# Autodesk Inventor assembly: Carriage_Link_COG
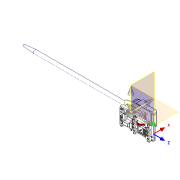
[picture p0: Inventor's stored thumbnail of the model, 180x180]
Saved by Autodesk Inventor 2022 (Build 260153000, 153)
## iProperties
Created: 2022-10-18
Part Number: Carriage_Link_COG
Document SubType Name: Assembly
Designer: alexw
Mass: 599.264 g
Surface Area: 1993.78 cm^2
Volume: 535.454 cm^3
Density: 1.11917 g/cm^3
Author: alexw
## Documents named in this file (22)
- C:\Users\alexw\Documents\Inventor\Projects\03_CurrentProjects\MasterThesis\PSM_V1_Rillenkugellager\COG\Carriage_Link_COG.iam
- C:\Users\alexw\Documents\Inventor\Projects\03_CurrentProjects\MasterThesis\PSM_V1_Rillenkugellager\Ueberarbeiteter DaVincikopf\Fuehrungsgrundplatte_V3.ipt
- C:\Users\alexw\Documents\Inventor\Projects\03_CurrentProjects\MasterThesis\PSM_V1_Rillenkugellager\Ueberarbeiteter DaVincikopf\JX BLS-HV7146MG.iam
- C:\Users\alexw\Documents\Inventor\Projects\03_CurrentProjects\MasterThesis\PSM_V1_Rillenkugellager\Ueberarbeiteter DaVincikopf\Op_dev_gehäuse.ipt
- C:\Users\alexw\Documents\Inventor\Projects\03_CurrentProjects\MasterThesis\PSM_V1_Rillenkugellager\Ueberarbeiteter DaVincikopf\Op_dev_stange.ipt
- C:\Users\alexw\Documents\Inventor\Projects\03_CurrentProjects\MasterThesis\PSM_V1_Rillenkugellager\Ueberarbeiteter DaVincikopf\Oberteil_servoplatte.ipt
- C:\Users\alexw\Documents\Inventor\Projects\03_CurrentProjects\MasterThesis\PSM_V1_Rillenkugellager\ContentCenter\de-DE\ISO 4762(2)\ISO 4762 - M4 x 30ISO.ipt
- C:\Users\alexw\Documents\Inventor\Projects\03_CurrentProjects\MasterThesis\PSM_V1_Rillenkugellager\ContentCenter\de-DE\ISO 4762(2)\ISO 4762 - M3 x 12ISO.ipt
- C:\Users\alexw\Documents\Inventor\Projects\03_CurrentProjects\MasterThesis\PSM_V1_Rillenkugellager\Ueberarbeiteter DaVincikopf\daVinciTool_Aufnahme.ipt
- C:\Users\alexw\Documents\Inventor\Projects\03_CurrentProjects\MasterThesis\PSM_V1_Rillenkugellager\Ueberarbeiteter DaVincikopf\daVinciTool_Aufnahme_ClutchPart.ipt
- C:\Users\alexw\Documents\Inventor\Projects\03_CurrentProjects\MasterThesis\PSM_V1_Rillenkugellager\Ueberarbeiteter DaVincikopf\daVincihead_Sled_ToolAufnahmeBuegel.ipt
- C:\Users\alexw\Documents\Inventor\Projects\03_CurrentProjects\MasterThesis\PSM_V1_Rillenkugellager\Ueberarbeiteter DaVincikopf\daVincihead_Sled_ToolAufnahmeBuegel_38mm.ipt
- C:\Users\alexw\Documents\Inventor\Projects\03_CurrentProjects\MasterThesis\PSM_V1_Rillenkugellager\Ueberarbeiteter DaVincikopf\3mmSchaft_50m.ipt
- C:\Users\alexw\Documents\Inventor\Projects\03_CurrentProjects\MasterThesis\PSM_V1_Rillenkugellager\Ueberarbeiteter DaVincikopf\3mmSchaft_63mm.ipt
- C:\Users\alexw\Documents\Inventor\Projects\03_CurrentProjects\MasterThesis\PSM_V1_Rillenkugellager\Ueberarbeiteter DaVincikopf\Fuehrungsrollen_Assembly.iam
- C:\Users\alexw\Documents\Inventor\Projects\03_CurrentProjects\MasterThesis\PSM_V1_Rillenkugellager\ContentCenter\de-DE\ISO 4762(2)\ISO 4762 - M3 x 10ISO.ipt
- C:\Users\alexw\Documents\Inventor\Projects\03_CurrentProjects\MasterThesis\PSM_V1_Rillenkugellager\Maschinenbauteil\spur_gear_1_30_6_6.ipt
- C:\Users\alexw\Documents\Inventor\Projects\03_CurrentProjects\MasterThesis\PSM_V1_Rillenkugellager\Ueberarbeiteter DaVincikopf\daVinciHead_HITEC_Assembly.iam
- C:\Users\alexw\Documents\Inventor\Projects\03_CurrentProjects\MasterThesis\PSM_V1_Rillenkugellager\Ueberarbeiteter DaVincikopf\Anpresspinns_Assembly.iam
- C:\Users\alexw\Documents\Inventor\Projects\03_CurrentProjects\MasterThesis\PSM_V1_Rillenkugellager\ContentCenter\de-DE\ISO 4762(2)\ISO 4762 - M4 x 12ISO.ipt
- C:\Users\alexw\Documents\Inventor\Projects\03_CurrentProjects\MasterThesis\PSM_V1_Rillenkugellager\ContentCenter\de-DE\ISO 10642(1)\ISO 10642 - M3 x  8.ipt
- C:\Users\alexw\Documents\Inventor\Projects\03_CurrentProjects\MasterThesis\PSM_V1_Rillenkugellager\ContentCenter\de-DE\ISO 4762(2)\ISO 4762 - M3 x 8ISO.ipt
## Components (46 placed, 21 different names)
1. Fuehrungsgrundplatte_V3:1 — Passend:95, Winkel:1, Passend:97
2. JX BLS-HV7146MG:1 [sub-assembly]
3. Op_dev_gehäuse:1
4. Op_dev_stange:1
5. Oberteil_servoplatte:1
6. ISO 4762 M4 x 30:1
7. ISO 4762 M4 x 30:2
8. ISO 4762 M3 x 12:1
9. ISO 4762 M3 x 12:2
10. ISO 4762 M3 x 12:3
11. ISO 4762 M3 x 12:4
12. daVinciTool_Aufnahme:1
13. daVinciTool_Aufnahme_ClutchPart:1
14. daVincihead_Sled_ToolAufnahmeBuegel:1 — Passend:96
15. daVincihead_Sled_ToolAufnahmeBuegel_38mm:1
16. 3mmSchaft_50m:1
17. 3mmSchaft_63mm:1
18. ISO 4762 M3 x 12:5
19. ISO 4762 M3 x 12:6
20. ISO 4762 M3 x 12:7
21. ISO 4762 M3 x 12:8
22. Fuehrungsrollen_Assembly:1 [sub-assembly]
23. Fuehrungsrollen_Assembly:2 [sub-assembly]
24. Fuehrungsrollen_Assembly:3 [sub-assembly]
25. ISO 4762 M3 x 10:1
26. ISO 4762 M3 x 10:2
27. ISO 4762 M3 x 10:3
28. ISO 4762 M3 x 10:4
29. ISO 4762 M3 x 10:5
30. ISO 4762 M3 x 10:6
31. spur_gear_1_30_6_6:1
32. daVinciHead_HITEC_Assembly:1 [sub-assembly]
33. daVinciHead_HITEC_Assembly:2 [sub-assembly]
34. daVinciHead_HITEC_Assembly:3 [sub-assembly]
35. daVinciHead_HITEC_Assembly:4 [sub-assembly]
36. Anpresspinns_Assembly:1 [sub-assembly]
37. Anpresspinns_Assembly:2 [sub-assembly]
38. Anpresspinns_Assembly:3 [sub-assembly]
39. Anpresspinns_Assembly:4 [sub-assembly]
40. ISO 4762 M4 x 12:1
41. 3mmSchaft_63mm:2
42. ISO 10642 M3x8:1
43. ISO 4762 M3 x 8:1
44. ISO 4762 M3 x 8:2
45. ISO 4762 M3 x 8:3
46. ISO 4762 M3 x 8:4
## Relationships (104: Mate 97, Flush 5, RevoluteJoint 1, Angle 1)
- [Flush] (-5 mm): Fuehrungsgrundplatte_V3:1 ↔ JX BLS-HV7146MG:1
- [Mate]: Fuehrungsgrundplatte_V3:1 ↔ JX BLS-HV7146MG:1
- [Mate]: Fuehrungsgrundplatte_V3:1 ↔ JX BLS-HV7146MG:1
- [RevoluteJoint]: Op_dev_gehäuse:1 ↔ Op_dev_stange:1
- [Mate]: Fuehrungsgrundplatte_V3:1 ↔ Oberteil_servoplatte:1
- [Flush]: Fuehrungsgrundplatte_V3:1 ↔ Oberteil_servoplatte:1
- [Mate]: Fuehrungsgrundplatte_V3:1 ↔ ISO 4762 M4 x 30:1
- [Mate]: Fuehrungsgrundplatte_V3:1 ↔ ISO 4762 M4 x 30:2
- [Mate]: Oberteil_servoplatte:1 ↔ ISO 4762 M3 x 12:1
- [Mate]: Oberteil_servoplatte:1 ↔ ISO 4762 M3 x 12:1
- [Mate]: Oberteil_servoplatte:1 ↔ ISO 4762 M3 x 12:2
- [Mate]: Oberteil_servoplatte:1 ↔ ISO 4762 M3 x 12:2
- [Mate]: Oberteil_servoplatte:1 ↔ ISO 4762 M3 x 12:3
- [Mate]: Oberteil_servoplatte:1 ↔ ISO 4762 M3 x 12:3
- [Mate]: Oberteil_servoplatte:1 ↔ ISO 4762 M3 x 12:4
- [Mate]: Oberteil_servoplatte:1 ↔ ISO 4762 M3 x 12:4
- [Mate] (-6.043 mm): Op_dev_gehäuse:1 ↔ daVinciTool_Aufnahme:1
- [Mate]: Op_dev_gehäuse:1 ↔ daVinciTool_Aufnahme:1
- [Flush]: daVinciTool_Aufnahme:1 ↔ daVinciTool_Aufnahme_ClutchPart:1
- [Mate]: Oberteil_servoplatte:1 ↔ daVincihead_Sled_ToolAufnahmeBuegel:1
- [Mate]: Oberteil_servoplatte:1 ↔ daVincihead_Sled_ToolAufnahmeBuegel_38mm:1
- [Mate]: daVincihead_Sled_ToolAufnahmeBuegel:1 ↔ 3mmSchaft_63mm:1
- [Mate]: daVincihead_Sled_ToolAufnahmeBuegel_38mm:1 ↔ 3mmSchaft_50m:1
- [Mate]: daVincihead_Sled_ToolAufnahmeBuegel_38mm:1 ↔ 3mmSchaft_50m:1
- [Mate]: daVinciTool_Aufnahme:1 ↔ 3mmSchaft_63mm:1
- [Mate]: Oberteil_servoplatte:1 ↔ daVinciTool_Aufnahme:1
- [Mate]: daVincihead_Sled_ToolAufnahmeBuegel_38mm:1 ↔ ISO 4762 M3 x 12:5
- [Mate]: Oberteil_servoplatte:1 ↔ ISO 4762 M3 x 12:5
- [Mate]: daVincihead_Sled_ToolAufnahmeBuegel_38mm:1 ↔ ISO 4762 M3 x 12:6
- [Mate]: Oberteil_servoplatte:1 ↔ ISO 4762 M3 x 12:6
- [Mate]: daVincihead_Sled_ToolAufnahmeBuegel:1 ↔ ISO 4762 M3 x 12:7
- [Mate]: Oberteil_servoplatte:1 ↔ ISO 4762 M3 x 12:7
- [Mate]: daVincihead_Sled_ToolAufnahmeBuegel:1 ↔ ISO 4762 M3 x 12:8
- [Mate]: Oberteil_servoplatte:1 ↔ ISO 4762 M3 x 12:8
- [Mate]: Oberteil_servoplatte:1 ↔ daVincihead_Sled_ToolAufnahmeBuegel_38mm:1
- [Mate]: Oberteil_servoplatte:1 ↔ daVincihead_Sled_ToolAufnahmeBuegel_38mm:1
- [Mate]: Oberteil_servoplatte:1 ↔ daVincihead_Sled_ToolAufnahmeBuegel:1
- [Mate]: Fuehrungsgrundplatte_V3:1 ↔ Fuehrungsrollen_Assembly:1
- [Mate]: Fuehrungsgrundplatte_V3:1 ↔ Fuehrungsrollen_Assembly:1
- [Mate]: Fuehrungsgrundplatte_V3:1 ↔ Fuehrungsrollen_Assembly:1
- [Mate]: Fuehrungsgrundplatte_V3:1 ↔ Fuehrungsrollen_Assembly:2
- [Mate]: Fuehrungsgrundplatte_V3:1 ↔ Fuehrungsrollen_Assembly:2
- [Mate]: Fuehrungsgrundplatte_V3:1 ↔ Fuehrungsrollen_Assembly:2
- [Mate]: Fuehrungsgrundplatte_V3:1 ↔ Fuehrungsrollen_Assembly:3
- [Mate]: Fuehrungsgrundplatte_V3:1 ↔ Fuehrungsrollen_Assembly:3
- [Mate]: Fuehrungsgrundplatte_V3:1 ↔ Fuehrungsrollen_Assembly:3
- [Mate]: Fuehrungsrollen_Assembly:1 ↔ ISO 4762 M3 x 10:1
- [Mate]: Fuehrungsrollen_Assembly:1 ↔ ISO 4762 M3 x 10:1
- [Mate]: Fuehrungsrollen_Assembly:1 ↔ ISO 4762 M3 x 10:2
- [Mate]: Fuehrungsrollen_Assembly:1 ↔ ISO 4762 M3 x 10:2
- [Mate]: Fuehrungsrollen_Assembly:2 ↔ ISO 4762 M3 x 10:3
- [Mate]: Fuehrungsrollen_Assembly:2 ↔ ISO 4762 M3 x 10:3
- [Mate]: Fuehrungsrollen_Assembly:2 ↔ ISO 4762 M3 x 10:4
- [Mate]: Fuehrungsrollen_Assembly:2 ↔ ISO 4762 M3 x 10:4
- [Mate]: Fuehrungsrollen_Assembly:3 ↔ ISO 4762 M3 x 10:5
- [Mate]: Fuehrungsrollen_Assembly:3 ↔ ISO 4762 M3 x 10:5
- [Mate]: Fuehrungsrollen_Assembly:3 ↔ ISO 4762 M3 x 10:6
- [Mate]: Fuehrungsrollen_Assembly:3 ↔ ISO 4762 M3 x 10:6
- [Mate]: JX BLS-HV7146MG:1 ↔ spur_gear_1_30_6_6:1
- [Mate]: JX BLS-HV7146MG:1 ↔ spur_gear_1_30_6_6:1
- [Mate]: JX BLS-HV7146MG:1 ↔ ISO 4762 M4 x 30:1
- [Mate]: JX BLS-HV7146MG:1 ↔ ISO 4762 M4 x 30:2
- [Mate]: Fuehrungsgrundplatte_V3:1 ↔ daVinciHead_HITEC_Assembly:2
- [Mate]: Fuehrungsgrundplatte_V3:1 ↔ daVinciHead_HITEC_Assembly:2
- [Mate]: Fuehrungsgrundplatte_V3:1 ↔ daVinciHead_HITEC_Assembly:2
- [Mate]: Fuehrungsgrundplatte_V3:1 ↔ daVinciHead_HITEC_Assembly:4
- [Mate]: Fuehrungsgrundplatte_V3:1 ↔ daVinciHead_HITEC_Assembly:4
- [Mate]: Fuehrungsgrundplatte_V3:1 ↔ daVinciHead_HITEC_Assembly:4
- [Mate]: Fuehrungsgrundplatte_V3:1 ↔ daVinciHead_HITEC_Assembly:1
- [Mate]: Fuehrungsgrundplatte_V3:1 ↔ daVinciHead_HITEC_Assembly:1
- [Mate]: Fuehrungsgrundplatte_V3:1 ↔ daVinciHead_HITEC_Assembly:1
- [Mate]: Fuehrungsgrundplatte_V3:1 ↔ daVinciHead_HITEC_Assembly:3
- [Mate]: Fuehrungsgrundplatte_V3:1 ↔ daVinciHead_HITEC_Assembly:3
- [Mate]: Fuehrungsgrundplatte_V3:1 ↔ daVinciHead_HITEC_Assembly:3
- [Mate]: daVinciTool_Aufnahme_ClutchPart:1 ↔ daVinciHead_HITEC_Assembly:2
- [Mate]: daVinciTool_Aufnahme_ClutchPart:1 ↔ daVinciHead_HITEC_Assembly:3
- [Mate]: Oberteil_servoplatte:1 ↔ Anpresspinns_Assembly:1
- [Mate]: daVinciTool_Aufnahme_ClutchPart:1 ↔ Anpresspinns_Assembly:1
- [Mate]: Oberteil_servoplatte:1 ↔ Anpresspinns_Assembly:2
- [Mate]: daVinciTool_Aufnahme_ClutchPart:1 ↔ Anpresspinns_Assembly:2
- [Mate]: Oberteil_servoplatte:1 ↔ Anpresspinns_Assembly:4
- [Mate]: Oberteil_servoplatte:1 ↔ Anpresspinns_Assembly:3
- [Mate]: daVinciTool_Aufnahme_ClutchPart:1 ↔ Anpresspinns_Assembly:4
- [Mate]: daVinciTool_Aufnahme_ClutchPart:1 ↔ Anpresspinns_Assembly:3
- [Mate]: Fuehrungsgrundplatte_V3:1 ↔ ISO 4762 M4 x 12:1
- [Mate]: JX BLS-HV7146MG:1 ↔ ISO 4762 M4 x 12:1
- [Mate]: Fuehrungsgrundplatte_V3:1 ↔ ISO 4762 M3 x 12:1
- [Flush]: daVincihead_Sled_ToolAufnahmeBuegel:1 ↔ 3mmSchaft_63mm:1
- [Mate]: daVinciTool_Aufnahme:1 ↔ 3mmSchaft_63mm:2
- [Flush]: daVincihead_Sled_ToolAufnahmeBuegel:1 ↔ 3mmSchaft_63mm:2
- [Mate]: Op_dev_gehäuse:1 ↔ daVinciTool_Aufnahme:1
- [Mate]: spur_gear_1_30_6_6:1 ↔ ISO 10642 M3x8:1
- [Mate]: Fuehrungsgrundplatte_V3:1 ↔ ISO 4762 M3 x 8:1
- [Mate]: Fuehrungsgrundplatte_V3:1 ↔ ISO 4762 M3 x 8:1
- [Mate]: Fuehrungsgrundplatte_V3:1 ↔ ISO 4762 M3 x 8:2
- [Mate]: Fuehrungsgrundplatte_V3:1 ↔ ISO 4762 M3 x 8:2
- [Mate]: Fuehrungsgrundplatte_V3:1 ↔ ISO 4762 M3 x 8:3
- [Mate]: Fuehrungsgrundplatte_V3:1 ↔ ISO 4762 M3 x 8:3
- [Mate]: Fuehrungsgrundplatte_V3:1 ↔ ISO 4762 M3 x 8:4
- [Mate]: Fuehrungsgrundplatte_V3:1 ↔ ISO 4762 M3 x 8:4
- Passend:95 [Mate]: Fuehrungsgrundplatte_V3:1
- Winkel:1 [Angle] (0 deg): Fuehrungsgrundplatte_V3:1
- Passend:96 [Mate]: daVincihead_Sled_ToolAufnahmeBuegel:1
- Passend:97 [Mate]: Fuehrungsgrundplatte_V3:1
## Named parameters: d53_d75 = 0 mm, d54_d76 = 52.289252 deg, d55_d88 = 0 mm, d56_d89 = 0 mm, d57_d116 = 0 mm, d58_d117 = 0 mm, d59_d118 = 0 mm, d60_d124 = 0 mm, d61_d125 = 0 mm, d62_d126 = 0 mm
